# Autodesk Inventor assembly: Assembly1タミヤダンパー 改
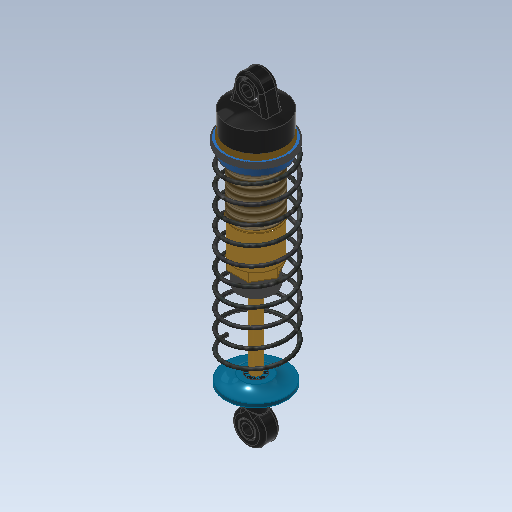
[picture p0: Inventor's stored thumbnail of the model, 512x512]
Saved by Autodesk Inventor 2020.2 (Build 242310000, 310)
## iProperties
Created: 2018-12-12
Part Number: Assembly1タミヤダンパー 改
Material: 一般
Document SubType Name: Assembly
Designer: 杉本　賢二郎
Mass: 34.6227 g
Surface Area: 82.5454 cm^2
Volume: 6.186 cm^3
Density: 5.59694 g/cm^3
Author: 杉本　賢二郎
## Documents named in this file (5)
- C:\Users\aoyam\Desktop\SRDC_local\Inventor\二年機\Geminiβ\汎用部品\ダンパー\Assembly1タミヤダンパー_リア.iam
- C:\Users\aoyam\Desktop\SRDC_local\Inventor\二年機\Geminiβ\汎用部品\ダンパー\Assembly2タミヤダンパー　下.iam
- C:\Users\aoyam\Desktop\SRDC_local\Inventor\二年機\Geminiβ\汎用部品\ダンパー\Assembly2タミヤダンパー　上.iam
- C:\Users\aoyam\Desktop\SRDC_local\Inventor\二年機\Geminiβ\汎用部品\ダンパー\タミヤダンパー部品9 (1).ipt
- C:\Users\aoyam\Desktop\SRDC_local\Inventor\二年機\Geminiβ\汎用部品\ダンパー\タミヤダンパー部品10_リアバネ.ipt
## Components (4 placed, 4 different names)
1. Assembly2タミヤダンパー　下:1 [sub-assembly] — 円柱状:1, フラッシュ:1, 挿入:1
2. Assembly2タミヤダンパー　上:1 [sub-assembly] — 円柱状:1, フラッシュ:1
3. タミヤダンパー部品9 (1):1 — 挿入:1
4. タミヤダンパー部品10_リアバネ:1
## Relationships (3: CylindricalJoint 1, Flush 1, Insert 1)
- 円柱状:1 [CylindricalJoint]: Assembly2タミヤダンパー　下:1 ↔ Assembly2タミヤダンパー　上:1
- フラッシュ:1 [Flush]: Assembly2タミヤダンパー　下:1 ↔ Assembly2タミヤダンパー　上:1
- 挿入:1 [Insert]: Assembly2タミヤダンパー　下:1 ↔ タミヤダンパー部品9 (1):1
